# Autodesk Inventor assembly: Assembly_Single_Depth
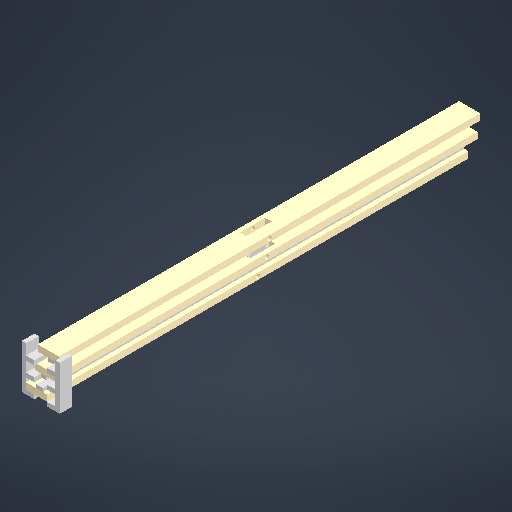
[picture p0: Inventor's stored thumbnail of the model, 512x512]
Saved by Autodesk Inventor 2026.1 (Build 301233020, 233B)
## iProperties
Created: 2026-03-11
Part Number: Assembly_Single_Depth
Document SubType Name: Assembly
Designer: elaij
Author: elaij
## Documents named in this file (6)
- C:\Users\elaij\OneDrive\Documents\MD Project 314\CAD_Concepts\Assembly_Single_Depth.iam
- C:\Users\elaij\OneDrive\Documents\MD Project 314\CAD_Concepts\Assembly_Dumb.iam
- C:\Users\elaij\OneDrive\Documents\MD Project 314\CAD_Concepts\Layer.ipt
- C:\Users\elaij\OneDrive\Documents\MD Project 314\CAD_Concepts\Rack.ipt
- C:\Users\elaij\OneDrive\Documents\MD Project 314\CAD_Concepts\Guide_Basic.ipt
- C:\Users\elaij\OneDrive\Documents\MD Project 314\CAD_Concepts\Gear_Basic.ipt
## Components (9 placed, 5 different names)
1. Assembly_Dumb:2 [sub-assembly] — Flush:6, Mate:8, Rotation/Translation:1, Rotation/Translation:2
2. Layer:1 — Mate:3, Flush:5, Flush:8, Flush:11, Mate:9
3. Rack:1 — Mate:3, Flush:5, Flush:6, Flush:8, Flush:11
4. Guide_Basic:1 — Mate:4, Flush:12, Flush:15, Mate:8, Flush:17, Flush:19, Mate:14, Flush:21, Flush:22
5. Guide_Basic:2 — Mate:14, Flush:21, Flush:22, Mate:15, Mate:16, Flush:23, Mate:17
6. Guide_Basic:3 — Mate:4, Flush:12, Flush:15, Mate:9
7. Layer:2 — Mate:15, Mate:16, Flush:23
8. Rack:2 — Rotation/Translation:2
9. Gear_Basic:1 — Drive, Rotation/Translation:1
## Relationships (27: Mate 12, Flush 12, RelateRotateTranslate 2, Angle 1)
- Mate:3: Layer:1 ↔ Rack:1
- Flush:5: Layer:1 ↔ Rack:1
- Flush:6: Assembly_Dumb:2 ↔ Rack:1
- Flush:8: Layer:1 ↔ Rack:1
- Flush:11 (-10 mm): Layer:1 ↔ Rack:1
- Mate:4: Guide_Basic:1 ↔ Guide_Basic:3
- Flush:12: Guide_Basic:1 ↔ Guide_Basic:3
- Flush:15: Guide_Basic:1 ↔ Guide_Basic:3
- Mate:8: Assembly_Dumb:2 ↔ Guide_Basic:1
- Mate:9: Layer:1 ↔ Guide_Basic:3
- Flush:17: Guide_Basic:1
- Flush:19: Guide_Basic:1
- [Mate]: Layer:2 ↔ Rack:2
- [Flush]: Layer:2 ↔ Rack:2
- [Mate]: Layer:2 ↔ Gear_Basic:1
- [Mate]: Layer:2 ↔ Gear_Basic:1
- [Mate]: Layer:2 ↔ Rack:2
- Drive [Angle] (720 deg): Gear_Basic:1
- Mate:14: Guide_Basic:1 ↔ Guide_Basic:2
- Flush:21: Guide_Basic:1 ↔ Guide_Basic:2
- Flush:22: Guide_Basic:1 ↔ Guide_Basic:2
- Mate:15: Guide_Basic:2 ↔ Layer:2
- Mate:16: Guide_Basic:2 ↔ Layer:2
- Flush:23: Guide_Basic:2 ↔ Layer:2
- Mate:17: Guide_Basic:2
- Rotation/Translation:1 [RelateRotateTranslate] (100 mm): Assembly_Dumb:2 ↔ Gear_Basic:1
- Rotation/Translation:2 [RelateRotateTranslate] (100 mm): Assembly_Dumb:2 ↔ Rack:2
## Named parameters: d52_d1 = 0 mm, d53_d2 = 0 mm
